# Autodesk Inventor assembly: nd
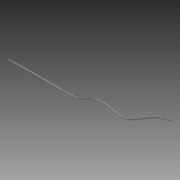
[picture p0: Inventor's stored thumbnail of the model, 180x180]
Saved by Autodesk Inventor 2015 (Build 190159000, 159)
## iProperties
Created: 2014-07-02
Part Number: nd
Document SubType Name: Assembly
Designer: peter
Author: peter
## Documents named in this file (67)
- C:\Users\peter\Documents\nd.iam
- C:\Users\peter\Documents\nd-1.ipt
- C:\Users\peter\Documents\nd-2.ipt
- C:\Users\peter\Documents\nd-3.ipt
- C:\Users\peter\Documents\nd-4.ipt
- C:\Users\peter\Documents\nd-5.ipt
- C:\Users\peter\Documents\nd-6.ipt
- C:\Users\peter\Documents\nd-7.ipt
- C:\Users\peter\Documents\nd-8.ipt
- C:\Users\peter\Documents\nd-9.ipt
- C:\Users\peter\Documents\nd-10.ipt
- C:\Users\peter\Documents\nd-11.ipt
- C:\Users\peter\Documents\nd-12.ipt
- C:\Users\peter\Documents\nd-13.ipt
- C:\Users\peter\Documents\nd-14.ipt
- C:\Users\peter\Documents\nd-15.ipt
- C:\Users\peter\Documents\nd-16.ipt
- C:\Users\peter\Documents\nd-1_MIR.ipt
- C:\Users\peter\Documents\nd-2_MIR.ipt
- C:\Users\peter\Documents\nd-3_MIR.ipt
- C:\Users\peter\Documents\nd-4_MIR.ipt
- C:\Users\peter\Documents\nd-5_MIR.ipt
- C:\Users\peter\Documents\nd-6_MIR.ipt
- C:\Users\peter\Documents\nd-7_MIR.ipt
- C:\Users\peter\Documents\nd-8_MIR.ipt
- C:\Users\peter\Documents\nd-9_MIR.ipt
- C:\Users\peter\Documents\nd-10_MIR.ipt
- C:\Users\peter\Documents\nd-11_MIR.ipt
- C:\Users\peter\Documents\nd-12_MIR.ipt
- C:\Users\peter\Documents\nd-13_MIR.ipt
- C:\Users\peter\Documents\nd-14_MIR.ipt
- C:\Users\peter\Documents\nd-15_MIR.ipt
- C:\Users\peter\Documents\nd-16_MIR.ipt
- C:\Users\peter\Documents\nd-a.ipt
- C:\Users\peter\Documents\nd-b.ipt
- C:\Users\peter\Documents\nd-c.ipt
- C:\Users\peter\Documents\nd-d.ipt
- C:\Users\peter\Documents\nd-e.ipt
- C:\Users\peter\Documents\nd-f.ipt
- C:\Users\peter\Documents\nd-g.ipt
- C:\Users\peter\Documents\nd-h.ipt
- C:\Users\peter\Documents\nd-i.ipt
- C:\Users\peter\Documents\nd-j.ipt
- C:\Users\peter\Documents\nd-k.ipt
- C:\Users\peter\Documents\nd-l.ipt
- C:\Users\peter\Documents\nd-m.ipt
- C:\Users\peter\Documents\nd-n.ipt
- C:\Users\peter\Documents\nd-o.ipt
- C:\Users\peter\Documents\nd-p.ipt
- C:\Users\peter\Documents\nd-17.ipt
- C:\Users\peter\Documents\nd-17_MIR.ipt
- C:\Users\peter\Documents\nd-a_MIR1.ipt
- C:\Users\peter\Documents\nd-b_MIR.ipt
- C:\Users\peter\Documents\nd-c_MIR.ipt
- C:\Users\peter\Documents\nd-d_MIR.ipt
- C:\Users\peter\Documents\nd-e_MIR.ipt
- C:\Users\peter\Documents\nd-f_MIR.ipt
- C:\Users\peter\Documents\nd-g_MIR.ipt
- C:\Users\peter\Documents\nd-h_MIR.ipt
- C:\Users\peter\Documents\nd-i_MIR.ipt
- C:\Users\peter\Documents\nd-j_MIR.ipt
- C:\Users\peter\Documents\nd-k_MIR.ipt
- C:\Users\peter\Documents\nd-l_MIR.ipt
- C:\Users\peter\Documents\nd-m_MIR.ipt
- C:\Users\peter\Documents\nd-n_MIR.ipt
- C:\Users\peter\Documents\nd-o_MIR.ipt
- C:\Users\peter\Documents\nd-p_MIR.ipt
## Components (66 placed, 66 different names)
1. nd-1:1 — Mate:1, Rigid:2
2. nd-2:1 — Mate:1, Mate:2, Rigid:2, Rigid:3
3. nd-3:1 — Mate:2, Mate:3, Rigid:3, Rigid:4
4. nd-4:1 — Mate:3, Mate:4, Rigid:1, Rigid:4
5. nd-5:1 — Mate:4, Mate:5, Rigid:1, Rigid:5
6. nd-6:1 — Mate:5, Rigid:5, Rigid:6
7. nd-7:1 — Rigid:6, Rigid:7
8. nd-8:1 — Rigid:7, Rigid:8
9. nd-9:1 — Rigid:8, Rigid:9
10. nd-10:1 — Rigid:9, Rigid:10
11. nd-11:1 — Rigid:10, Rigid:11
12. nd-12:1 — Rigid:11, Rigid:12
13. nd-13:1 — Rigid:12, Rigid:13
14. nd-14:1 — Rigid:13, Rigid:14
15. nd-15:1 — Rigid:14, Rigid:15
16. nd-16:1 — Rigid:15
17. nd-1_MIR:1 — Mate:6, Rigid:16, Rigid:31
18. nd-2_MIR:1 — Mate:6, Mate:7, Rigid:16, Rigid:17
19. nd-3_MIR:1 — Mate:7, Mate:8, Rigid:17, Rigid:18
20. nd-4_MIR:1 — Mate:8, Mate:9, Rigid:18, Rigid:19
21. nd-5_MIR:1 — Mate:9, Mate:10, Rigid:19, Rigid:20
22. nd-6_MIR:1 — Mate:10, Rigid:20, Rigid:21
23. nd-7_MIR:1 — Rigid:21, Rigid:22
24. nd-8_MIR:1 — Rigid:22, Rigid:23
25. nd-9_MIR:1 — Rigid:23, Rigid:24
26. nd-10_MIR:1 — Rigid:24, Rigid:25
27. nd-11_MIR:1 — Rigid:25, Rigid:26
28. nd-12_MIR:1 — Rigid:26, Rigid:27
29. nd-13_MIR:1 — Rigid:27, Rigid:28
30. nd-14_MIR:1 — Rigid:28, Rigid:29
31. nd-15_MIR:1 — Rigid:29, Rigid:30
32. nd-16_MIR:1 — Rigid:30
33. nd-a:1 — Rigid:31, Rigid:34
34. nd-b:3 — Rigid:34, Rigid:35
35. nd-c:1 — Rigid:35, Rigid:36
36. nd-d:1 — Rigid:36, Rigid:37
37. nd-e:1 — Rigid:37, Rigid:38
38. nd-f:1 — Rigid:38, Rigid:39
39. nd-g:1 — Rigid:39, Rigid:40
40. nd-h:1 — Rigid:40, Rigid:41
41. nd-i:1 — Rigid:41, Rigid:42
42. nd-j:1 — Rigid:42, Rigid:43
43. nd-k:1 — Rigid:43, Rigid:44
44. nd-l:1 — Rigid:44, Rigid:45
45. nd-m:1 — Rigid:45, Rigid:46
46. nd-n:1 — Rigid:46, Rigid:47
47. nd-o:1 — Rigid:47, Rigid:48
48. nd-p:1 — Rigid:48, Rigid:49
49. nd-17:1 — Rigid:49
50. nd-17_MIR:1 — Rigid:65
51. nd-a_MIR1:1 — Rigid:50
52. nd-b_MIR:1 — Rigid:50, Rigid:51
53. nd-c_MIR:1 — Rigid:51, Rigid:52
54. nd-d_MIR:1 — Rigid:52, Rigid:53
55. nd-e_MIR:1 — Rigid:53, Rigid:54
56. nd-f_MIR:1 — Rigid:54, Rigid:55
57. nd-g_MIR:1 — Rigid:55, Rigid:56
58. nd-h_MIR:1 — Rigid:56, Rigid:57
59. nd-i_MIR:1 — Rigid:57, Rigid:58
60. nd-j_MIR:1 — Rigid:58, Rigid:59
61. nd-k_MIR:1 — Rigid:59, Rigid:60
62. nd-l_MIR:1 — Rigid:60, Rigid:61
63. nd-m_MIR:1 — Rigid:61, Rigid:62
64. nd-n_MIR:1 — Rigid:62, Rigid:63
65. nd-o_MIR:1 — Rigid:63, Rigid:64
66. nd-p_MIR:1 — Rigid:64, Rigid:65
## Relationships (73: WeldJoint 63, Mate 10)
- Mate:1: nd-1:1 ↔ nd-2:1
- Mate:2: nd-2:1 ↔ nd-3:1
- Mate:3: nd-3:1 ↔ nd-4:1
- Mate:4: nd-4:1 ↔ nd-5:1
- Mate:5: nd-5:1 ↔ nd-6:1
- Rigid:1 [WeldJoint]: nd-4:1 ↔ nd-5:1
- Rigid:2 [WeldJoint]: nd-1:1 ↔ nd-2:1
- Rigid:3 [WeldJoint]: nd-2:1 ↔ nd-3:1
- Rigid:4 [WeldJoint]: nd-3:1 ↔ nd-4:1
- Rigid:5 [WeldJoint]: nd-5:1 ↔ nd-6:1
- Rigid:6 [WeldJoint]: nd-6:1 ↔ nd-7:1
- Rigid:7 [WeldJoint]: nd-7:1 ↔ nd-8:1
- Rigid:8 [WeldJoint]: nd-8:1 ↔ nd-9:1
- Rigid:9 [WeldJoint]: nd-9:1 ↔ nd-10:1
- Rigid:10 [WeldJoint]: nd-10:1 ↔ nd-11:1
- Rigid:11 [WeldJoint]: nd-11:1 ↔ nd-12:1
- Rigid:12 [WeldJoint]: nd-12:1 ↔ nd-13:1
- Rigid:13 [WeldJoint]: nd-13:1 ↔ nd-14:1
- Rigid:14 [WeldJoint]: nd-14:1 ↔ nd-15:1
- Rigid:15 [WeldJoint]: nd-15:1 ↔ nd-16:1
- Mate:6: nd-1_MIR:1 ↔ nd-2_MIR:1
- Mate:7: nd-2_MIR:1 ↔ nd-3_MIR:1
- Mate:8: nd-3_MIR:1 ↔ nd-4_MIR:1
- Mate:9: nd-4_MIR:1 ↔ nd-5_MIR:1
- Mate:10: nd-5_MIR:1 ↔ nd-6_MIR:1
- Rigid:16 [WeldJoint]: nd-1_MIR:1 ↔ nd-2_MIR:1
- Rigid:17 [WeldJoint]: nd-2_MIR:1 ↔ nd-3_MIR:1
- Rigid:18 [WeldJoint]: nd-3_MIR:1 ↔ nd-4_MIR:1
- Rigid:19 [WeldJoint]: nd-4_MIR:1 ↔ nd-5_MIR:1
- Rigid:20 [WeldJoint]: nd-5_MIR:1 ↔ nd-6_MIR:1
- Rigid:21 [WeldJoint]: nd-6_MIR:1 ↔ nd-7_MIR:1
- Rigid:22 [WeldJoint]: nd-7_MIR:1 ↔ nd-8_MIR:1
- Rigid:23 [WeldJoint]: nd-8_MIR:1 ↔ nd-9_MIR:1
- Rigid:24 [WeldJoint]: nd-9_MIR:1 ↔ nd-10_MIR:1
- Rigid:25 [WeldJoint]: nd-10_MIR:1 ↔ nd-11_MIR:1
- Rigid:26 [WeldJoint]: nd-11_MIR:1 ↔ nd-12_MIR:1
- Rigid:27 [WeldJoint]: nd-12_MIR:1 ↔ nd-13_MIR:1
- Rigid:28 [WeldJoint]: nd-13_MIR:1 ↔ nd-14_MIR:1
- Rigid:29 [WeldJoint]: nd-14_MIR:1 ↔ nd-15_MIR:1
- Rigid:30 [WeldJoint]: nd-15_MIR:1 ↔ nd-16_MIR:1
- Rigid:31 [WeldJoint]: nd-1_MIR:1 ↔ nd-a:1
- Rigid:34 [WeldJoint]: nd-a:1 ↔ nd-b:3
- Rigid:35 [WeldJoint]: nd-b:3 ↔ nd-c:1
- Rigid:36 [WeldJoint]: nd-c:1 ↔ nd-d:1
- Rigid:37 [WeldJoint]: nd-d:1 ↔ nd-e:1
- Rigid:38 [WeldJoint]: nd-e:1 ↔ nd-f:1
- Rigid:39 [WeldJoint]: nd-f:1 ↔ nd-g:1
- Rigid:40 [WeldJoint]: nd-g:1 ↔ nd-h:1
- Rigid:41 [WeldJoint]: nd-h:1 ↔ nd-i:1
- Rigid:42 [WeldJoint]: nd-i:1 ↔ nd-j:1
- Rigid:43 [WeldJoint]: nd-j:1 ↔ nd-k:1
- Rigid:44 [WeldJoint]: nd-k:1 ↔ nd-l:1
- Rigid:45 [WeldJoint]: nd-l:1 ↔ nd-m:1
- Rigid:46 [WeldJoint]: nd-m:1 ↔ nd-n:1
- Rigid:47 [WeldJoint]: nd-n:1 ↔ nd-o:1
- Rigid:48 [WeldJoint]: nd-o:1 ↔ nd-p:1
- Rigid:49 [WeldJoint]: nd-p:1 ↔ nd-17:1
- Rigid:50 [WeldJoint]: nd-a_MIR1:1 ↔ nd-b_MIR:1
- Rigid:51 [WeldJoint]: nd-b_MIR:1 ↔ nd-c_MIR:1
- Rigid:52 [WeldJoint]: nd-c_MIR:1 ↔ nd-d_MIR:1
- Rigid:53 [WeldJoint]: nd-d_MIR:1 ↔ nd-e_MIR:1
- Rigid:54 [WeldJoint]: nd-e_MIR:1 ↔ nd-f_MIR:1
- Rigid:55 [WeldJoint]: nd-f_MIR:1 ↔ nd-g_MIR:1
- Rigid:56 [WeldJoint]: nd-g_MIR:1 ↔ nd-h_MIR:1
- Rigid:57 [WeldJoint]: nd-h_MIR:1 ↔ nd-i_MIR:1
- Rigid:58 [WeldJoint]: nd-i_MIR:1 ↔ nd-j_MIR:1
- Rigid:59 [WeldJoint]: nd-j_MIR:1 ↔ nd-k_MIR:1
- Rigid:60 [WeldJoint]: nd-k_MIR:1 ↔ nd-l_MIR:1
- Rigid:61 [WeldJoint]: nd-l_MIR:1 ↔ nd-m_MIR:1
- Rigid:62 [WeldJoint]: nd-m_MIR:1 ↔ nd-n_MIR:1
- Rigid:63 [WeldJoint]: nd-n_MIR:1 ↔ nd-o_MIR:1
- Rigid:64 [WeldJoint]: nd-o_MIR:1 ↔ nd-p_MIR:1
- Rigid:65 [WeldJoint]: nd-17_MIR:1 ↔ nd-p_MIR:1
